# Autodesk Inventor assembly: Hot End Assembly
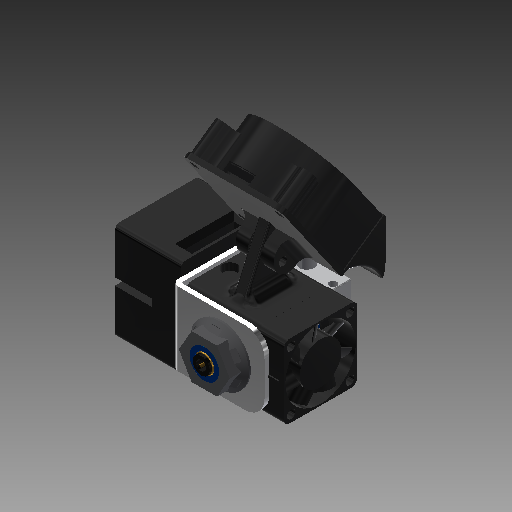
[picture p0: Inventor's stored thumbnail of the model, 512x512]
Saved by Autodesk Inventor 2019 (Build 230136000, 136)
## iProperties
Created: 2018-12-14
Part Number: Hot End Assembly
Document SubType Name: Assembly
Designer: Ax
Mass: 105.743 g
Surface Area: 661.515 cm^2
Volume: 82.9232 cm^3
Density: 1.27519 g/cm^3
Author: Ax
## Documents named in this file (10)
- C:\Users\Ax\Google Drive\Inventor\AX-01\Hot End Assembly.iam
- C:\Users\Ax\Google Drive\Inventor\Library\E3Dv6_1_75mm_Threaded_Heatsink .iam
- C:\Users\Ax\Google Drive\Inventor\Library\Layer_Fan_Mount.ipt
- C:\Users\Ax\Google Drive\Inventor\Library\30mm Fan.ipt
- C:\Users\Ax\Google Drive\Inventor\Library\blower_fan.ipt
- C:\Users\Ax\Google Drive\Inventor\AX-01\Hot End Mount.ipt
- C:\Users\Ax\Google Drive\Inventor\Library\Nylon Nut.ipt
- C:\Users\Ax\Google Drive\Inventor\AX-01\Electromagnet Block.ipt
- C:\Users\Ax\Google Drive\Inventor\AX-01\20-15 Electromagnet.ipt
- C:\Users\Ax\Google Drive\Inventor\AX-01\Heatsink_Fan_Fan Right.ipt
## Components (9 placed, 9 different names)
1. E3Dv6_1_75mm_Threaded_Heatsink :1 [sub-assembly] — Mate:1, Mate:2, Flush:1, Rigid:5
2. Layer_Fan_Mount:2 — Mate:9, Mate:10, Mate:11, Rigid:8
3. 30mm Fan:1 — Mate:17, Mate:18, Mate:19
4. blower_fan:2 — Mate:9, Mate:10, Mate:11
5. Hot End Mount:1 — Rigid:4, Rigid:5, Rigid:6, Rigid:7
6. Nylon Nut:1 — Rigid:6
7. Electromagnet Block:1 — Mate:15, Mate:16, Rigid:4
8. 20-15 Electromagnet:1 — Mate:15, Mate:16
9. Heatsink_Fan_Fan Right:1 — Rigid:7, Mate:17, Mate:18, Mate:19, Rigid:8
## Relationships (16: Mate 10, WeldJoint 5, Flush 1)
- Mate:1: E3Dv6_1_75mm_Threaded_Heatsink :1
- Mate:2: E3Dv6_1_75mm_Threaded_Heatsink :1
- Flush:1: E3Dv6_1_75mm_Threaded_Heatsink :1
- Mate:9: Layer_Fan_Mount:2 ↔ blower_fan:2
- Mate:10: Layer_Fan_Mount:2 ↔ blower_fan:2
- Mate:11: Layer_Fan_Mount:2 ↔ blower_fan:2
- Mate:15: Electromagnet Block:1 ↔ 20-15 Electromagnet:1
- Mate:16: Electromagnet Block:1 ↔ 20-15 Electromagnet:1
- Rigid:4 [WeldJoint]: Hot End Mount:1 ↔ Electromagnet Block:1
- Rigid:5 [WeldJoint]: E3Dv6_1_75mm_Threaded_Heatsink :1 ↔ Hot End Mount:1
- Rigid:6 [WeldJoint]: Hot End Mount:1 ↔ Nylon Nut:1
- Rigid:7 [WeldJoint]: Hot End Mount:1 ↔ Heatsink_Fan_Fan Right:1
- Mate:17: 30mm Fan:1 ↔ Heatsink_Fan_Fan Right:1
- Mate:18: 30mm Fan:1 ↔ Heatsink_Fan_Fan Right:1
- Mate:19: 30mm Fan:1 ↔ Heatsink_Fan_Fan Right:1
- Rigid:8 [WeldJoint]: Layer_Fan_Mount:2 ↔ Heatsink_Fan_Fan Right:1
